# Autodesk Inventor assembly: VexPro Ballshifter 3 stage
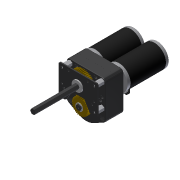
[picture p0: Inventor's stored thumbnail of the model, 180x180]
Saved by Autodesk Inventor 2013 (Build 170138000, 138)
## iProperties
Created: 2013-04-08
Part Number: VexPro Ballshifter 3 stage
Document SubType Name: Assembly
Designer: Niemitalo_Dan
Author: Niemitalo_Dan
## Documents named in this file (21)
- H:\Nemo\Documents\Robotics\COTS Parts\Ballshifter\VexPro Ballshifter 3 stage.iam
- H:\Nemo\Documents\Robotics\COTS Parts\Ballshifter\Ball Shifter Housing - Motor Side.ipt
- H:\Nemo\Documents\Robotics\COTS Parts\Bearings - VexPro\Flanged Bearing - 0.75in x 1.375in x .437in.ipt
- H:\Nemo\Documents\Robotics\COTS Parts\Bearings - VexPro\Flanged Bearing - 0.5in Round ID x 1.125in OD.ipt
- H:\Nemo\Documents\Robotics\COTS Parts\Ballshifter\Ball Shifter Housing - Output Side.ipt
- H:\Nemo\Documents\Robotics\COTS Parts\Bearings - VexPro\Flanged Bearing - 0.375in Round ID x 0.875in OD.ipt
- H:\Nemo\Documents\Robotics\COTS Parts\Ballshifter\Ballshifter 375 hex cluster shaft.ipt
- H:\Nemo\Documents\Robotics\COTS Parts\Gears - VexPro\Gear 20dp 375hex 24T Vex.ipt
- H:\Nemo\Documents\Robotics\COTS Parts\Gears - VexPro\Gear 20dp 375hex 40T Vex.ipt
- H:\Nemo\Documents\Robotics\COTS Parts\Ballshifter\CIM for Ballshifter.iam
- H:\Nemo\Documents\Robotics\COTS Parts\Fasteners\6-32 SHCS x250.ipt
- H:\Nemo\Documents\Robotics\COTS Parts\Ballshifter\Shifting Cylinder Mechanism for Ball Shifter.iam
- H:\Nemo\Documents\Robotics\COTS Parts\Ballshifter\Ball Shifter shifting shaft with gears 3 stage.iam
- H:\Nemo\Documents\Robotics\COTS Parts\Gears - VexPro\Gear 20dp 500hex 34T Vex.ipt
- H:\Nemo\Documents\Robotics\COTS Parts\Bearings - VexPro\Radial Bearing - 0.5in x 1.125in x .313in.ipt
- H:\Nemo\Documents\Robotics\COTS Parts\Fasteners\KlipRing for 500hex.ipt
- H:\Nemo\Documents\Robotics\COTS Parts\Ballshifter\Ball Shifter 3 Stage Standoff.ipt
- H:\Nemo\Documents\Robotics\COTS Parts\Ballshifter\Ball Shifter 3rd stage Output Shaft.ipt
- H:\Nemo\Documents\Robotics\COTS Parts\Ballshifter\Ball Shifter 3rd Stage Plate.ipt
- H:\Nemo\Documents\Robotics\COTS Parts\Gears - VexPro\Gear 20dp 500hex 50T Vex.ipt
- H:\Nemo\Documents\Robotics\COTS Parts\Bearings - VexPro\Flanged Bearing - 0.5in Hex ID x 1.125in OD.ipt
## Components (27 placed, 20 different names)
1. Ball Shifter Housing - Motor Side:1 — Insert:1, Mate:1, Mate:2, Insert:4, Insert:9, Mate:3, Insert:10, Mate:4, Mate:5, Mate:6, Mate:7, Mate:8, Mate:9, Mate:18
2. Ball Shifter Housing - Output Side:1 — Mate:1, Mate:2, Insert:3, Insert:5, Mate:5, Mate:9, Insert:12, Mate:12, Mate:13, Angle:4, Angle:5, Mate:14, Mate:15, Mate:16, Angle:6, Mate:17, Angle:7, Mate:19
3. Flanged Bearing - 0.75in x 1.375in x .437in:1 — Insert:3
4. Flanged Bearing - 0.5in Round ID x 1.125in OD:1 — Insert:1, Insert:2
5. Ball Shifter shifting shaft with gears 3 stage:1 [sub-assembly] — Insert:2, Mate:10, Angle:3, Mate:11, Insert:13
6. Flanged Bearing - 0.375in Round ID x 0.875in OD:1 — Insert:5
7. Flanged Bearing - 0.375in Round ID x 0.875in OD:2 — Insert:4, Insert:6, Insert:7
8. Ballshifter 375 hex cluster shaft:1 — Insert:6, Angle:1, Angle:2
9. Gear 20dp 375hex 24T Vex:1 — Insert:8, Angle:2
10. Gear 20dp 375hex 40T Vex:1 — Insert:7, Angle:1, Insert:8
11. CIM for Ballshifter:1 [sub-assembly] — Insert:10, Mate:4
12. CIM for Ballshifter:2 [sub-assembly] — Insert:9, Mate:3
13. 6-32 SHCS x250:1
14. 6-32 SHCS x250:2
15. Shifting Cylinder Mechanism for Ball Shifter:1 [sub-assembly] — Mate:6, Mate:7, Mate:8
16. Gear 20dp 500hex 34T Vex:1 — Mate:10, Angle:3, Mate:11
17. Radial Bearing - 0.5in x 1.125in x .313in:1 — Insert:12, Insert:15
18. KlipRing for 500hex:1 — Insert:13
19. Ball Shifter 3 Stage Standoff:1 — Mate:18, Angle:7, Mate:19
20. Ball Shifter 3 Stage Standoff:2 — Mate:16, Angle:6, Mate:17
21. Ball Shifter 3 Stage Standoff:3 — Angle:5, Mate:14, Mate:15, Mate:22
22. Ball Shifter 3 Stage Standoff:4 — Mate:12, Mate:13, Angle:4, Insert:16
23. Ball Shifter 3rd stage Output Shaft:1 — Insert:14, Insert:15, Mate:20, Angle:8
24. Ball Shifter 3rd Stage Plate:1 — Insert:16, Mate:22, Insert:17
25. KlipRing for 500hex:2 — Insert:14, Mate:21
26. Gear 20dp 500hex 50T Vex:1 — Mate:20, Angle:8, Mate:21
27. Flanged Bearing - 0.5in Hex ID x 1.125in OD:1 — Insert:17
## Relationships (46: Mate 22, Insert 16, Angle 8)
- Insert:1: Ball Shifter Housing - Motor Side:1 ↔ Flanged Bearing - 0.5in Round ID x 1.125in OD:1
- Insert:2: Flanged Bearing - 0.5in Round ID x 1.125in OD:1 ↔ Ball Shifter shifting shaft with gears 3 stage:1
- Mate:1: Ball Shifter Housing - Motor Side:1 ↔ Ball Shifter Housing - Output Side:1
- Mate:2: Ball Shifter Housing - Motor Side:1 ↔ Ball Shifter Housing - Output Side:1
- Insert:3: Ball Shifter Housing - Output Side:1 ↔ Flanged Bearing - 0.75in x 1.375in x .437in:1
- Insert:4: Ball Shifter Housing - Motor Side:1 ↔ Flanged Bearing - 0.375in Round ID x 0.875in OD:2
- Insert:5: Ball Shifter Housing - Output Side:1 ↔ Flanged Bearing - 0.375in Round ID x 0.875in OD:1
- Insert:6: Flanged Bearing - 0.375in Round ID x 0.875in OD:2 ↔ Ballshifter 375 hex cluster shaft:1
- Insert:7: Flanged Bearing - 0.375in Round ID x 0.875in OD:2 ↔ Gear 20dp 375hex 40T Vex:1
- Angle:1 (0 deg): Ballshifter 375 hex cluster shaft:1 ↔ Gear 20dp 375hex 40T Vex:1
- Insert:8 (1.5875 mm): Gear 20dp 375hex 24T Vex:1 ↔ Gear 20dp 375hex 40T Vex:1
- Angle:2 (0 deg): Ballshifter 375 hex cluster shaft:1 ↔ Gear 20dp 375hex 24T Vex:1
- Insert:9: Ball Shifter Housing - Motor Side:1 ↔ CIM for Ballshifter:2
- Mate:3: Ball Shifter Housing - Motor Side:1 ↔ CIM for Ballshifter:2
- Insert:10: Ball Shifter Housing - Motor Side:1 ↔ CIM for Ballshifter:1
- Mate:4: Ball Shifter Housing - Motor Side:1 ↔ CIM for Ballshifter:1
- Mate:5: Ball Shifter Housing - Motor Side:1 ↔ Ball Shifter Housing - Output Side:1
- Mate:6: Ball Shifter Housing - Motor Side:1 ↔ Shifting Cylinder Mechanism for Ball Shifter:1
- Mate:7: Ball Shifter Housing - Motor Side:1 ↔ Shifting Cylinder Mechanism for Ball Shifter:1
- Mate:8: Ball Shifter Housing - Motor Side:1 ↔ Shifting Cylinder Mechanism for Ball Shifter:1
- Mate:9: Ball Shifter Housing - Motor Side:1 ↔ Ball Shifter Housing - Output Side:1
- Mate:10: Ball Shifter shifting shaft with gears 3 stage:1 ↔ Gear 20dp 500hex 34T Vex:1
- Angle:3 (0 deg): Ball Shifter shifting shaft with gears 3 stage:1 ↔ Gear 20dp 500hex 34T Vex:1
- Mate:11: Ball Shifter shifting shaft with gears 3 stage:1 ↔ Gear 20dp 500hex 34T Vex:1
- Insert:12: Ball Shifter Housing - Output Side:1 ↔ Radial Bearing - 0.5in x 1.125in x .313in:1
- Insert:13: Ball Shifter shifting shaft with gears 3 stage:1 ↔ KlipRing for 500hex:1
- Mate:12: Ball Shifter Housing - Output Side:1 ↔ Ball Shifter 3 Stage Standoff:4
- Mate:13: Ball Shifter Housing - Output Side:1 ↔ Ball Shifter 3 Stage Standoff:4
- Angle:4 (0 deg): Ball Shifter Housing - Output Side:1 ↔ Ball Shifter 3 Stage Standoff:4
- Angle:5 (0 deg): Ball Shifter Housing - Output Side:1 ↔ Ball Shifter 3 Stage Standoff:3
- Mate:14: Ball Shifter Housing - Output Side:1 ↔ Ball Shifter 3 Stage Standoff:3
- Mate:15: Ball Shifter Housing - Output Side:1 ↔ Ball Shifter 3 Stage Standoff:3
- Mate:16: Ball Shifter Housing - Output Side:1 ↔ Ball Shifter 3 Stage Standoff:2
- Angle:6 (0 deg): Ball Shifter Housing - Output Side:1 ↔ Ball Shifter 3 Stage Standoff:2
- Mate:17: Ball Shifter Housing - Output Side:1 ↔ Ball Shifter 3 Stage Standoff:2
- Mate:18: Ball Shifter Housing - Motor Side:1 ↔ Ball Shifter 3 Stage Standoff:1
- Angle:7 (0 deg): Ball Shifter Housing - Output Side:1 ↔ Ball Shifter 3 Stage Standoff:1
- Mate:19: Ball Shifter Housing - Output Side:1 ↔ Ball Shifter 3 Stage Standoff:1
- Insert:14: Ball Shifter 3rd stage Output Shaft:1 ↔ KlipRing for 500hex:2
- Insert:15: Radial Bearing - 0.5in x 1.125in x .313in:1 ↔ Ball Shifter 3rd stage Output Shaft:1
- Mate:20: Ball Shifter 3rd stage Output Shaft:1 ↔ Gear 20dp 500hex 50T Vex:1
- Angle:8 (0 deg): Ball Shifter 3rd stage Output Shaft:1 ↔ Gear 20dp 500hex 50T Vex:1
- Mate:21: KlipRing for 500hex:2 ↔ Gear 20dp 500hex 50T Vex:1
- Insert:16: Ball Shifter 3 Stage Standoff:4 ↔ Ball Shifter 3rd Stage Plate:1
- Mate:22: Ball Shifter 3 Stage Standoff:3 ↔ Ball Shifter 3rd Stage Plate:1
- Insert:17: Ball Shifter 3rd Stage Plate:1 ↔ Flanged Bearing - 0.5in Hex ID x 1.125in OD:1
